# Autodesk Inventor assembly: Button Fixture Assembly
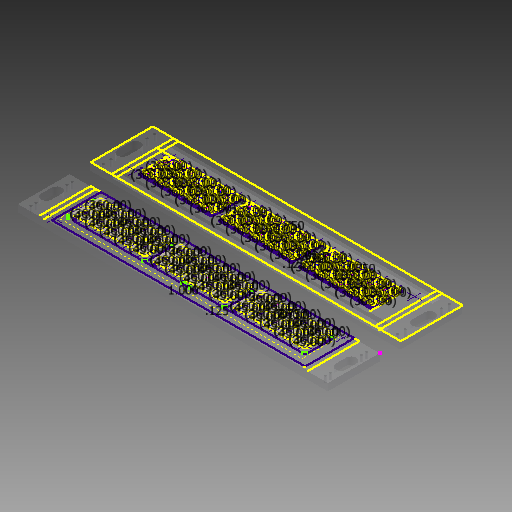
[picture p0: Inventor's stored thumbnail of the model, 512x512]
Saved by Autodesk Inventor 2018 (Build 220112000, 112)
## iProperties
Created: 2016-07-07
Part Number: Button Fixture Assembly
Document SubType Name: Assembly
Designer: Sam Clay
Author: Sam Clay
## Documents named in this file (3)
- Z:\enclosure\inventor\Button Fixture Assembly.iam
- Z:\enclosure\inventor\Button Fixture Base.ipt
- Z:\enclosure\inventor\Case Buttons CAM.ipt
## Components (61 placed, 2 different names)
1. Button Fixture Base:1 — Mate:9, Mate:10, Mate:11, Mate:12
2. Case Buttons CAM:9
3. Case Buttons CAM:10
4. Case Buttons CAM:11 — Mate:9
5. Case Buttons CAM:12
6. Case Buttons CAM:41
7. Case Buttons CAM:42
8. Case Buttons CAM:126
9. Case Buttons CAM:127
10. Case Buttons CAM:128
11. Case Buttons CAM:129
12. Case Buttons CAM:25
13. Case Buttons CAM:26
14. Case Buttons CAM:27
15. Case Buttons CAM:28
16. Case Buttons CAM:53
17. Case Buttons CAM:54
18. Case Buttons CAM:130
19. Case Buttons CAM:131
20. Case Buttons CAM:132
21. Case Buttons CAM:133
22. Case Buttons CAM:90
23. Case Buttons CAM:91
24. Case Buttons CAM:92
25. Case Buttons CAM:93
26. Case Buttons CAM:94
27. Case Buttons CAM:95
28. Case Buttons CAM:134
29. Case Buttons CAM:135
30. Case Buttons CAM:136
31. Case Buttons CAM:137
32. Case Buttons CAM:17 — Mate:10, Mate:11, Mate:12
33. Case Buttons CAM:18
34. Case Buttons CAM:19
35. Case Buttons CAM:20
36. Case Buttons CAM:64
37. Case Buttons CAM:65
38. Case Buttons CAM:138
39. Case Buttons CAM:139
40. Case Buttons CAM:140
41. Case Buttons CAM:141
42. Case Buttons CAM:29
43. Case Buttons CAM:30
44. Case Buttons CAM:31
45. Case Buttons CAM:32
46. Case Buttons CAM:76
47. Case Buttons CAM:77
48. Case Buttons CAM:142
49. Case Buttons CAM:143
50. Case Buttons CAM:144
51. Case Buttons CAM:145
52. Case Buttons CAM:108
53. Case Buttons CAM:109
54. Case Buttons CAM:110
55. Case Buttons CAM:111
56. Case Buttons CAM:112
57. Case Buttons CAM:113
58. Case Buttons CAM:146
59. Case Buttons CAM:147
60. Case Buttons CAM:148
61. Case Buttons CAM:149
## Component patterns: (3 elements), (3 elements), (10 elements, first: Case Buttons CAM:9), Component Pattern 3:2 (10 elements), Component Pattern 3:3 (10 elements), (10 elements, first: Case Buttons CAM:17), Component Pattern 4:2 (10 elements), Component Pattern 4:3 (10 elements)
## Relationships (4: Mate 4)
- Mate:9 (0.762 mm): Button Fixture Base:1 ↔ Case Buttons CAM:11
- Mate:10 (11.43 mm): Button Fixture Base:1 ↔ Case Buttons CAM:17
- Mate:11 (-25.4 mm): Button Fixture Base:1 ↔ Case Buttons CAM:17
- Mate:12 (-38.1 mm): Button Fixture Base:1 ↔ Case Buttons CAM:17
